# Autodesk Inventor assembly: Ventil
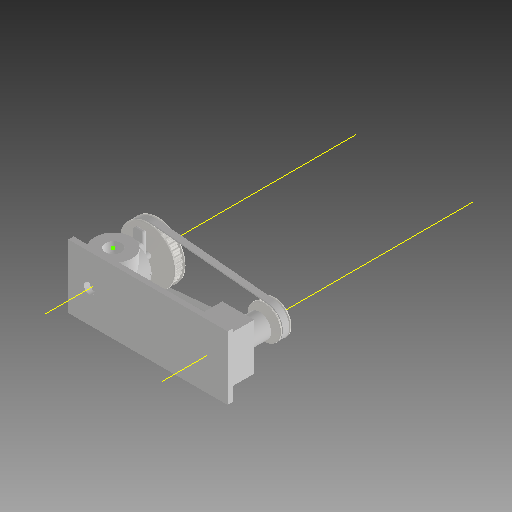
[picture p0: Inventor's stored thumbnail of the model, 512x512]
Saved by Autodesk Inventor 2021 (Build 250183000, 183)
## iProperties
Created: 2021-06-23
Part Number: Ventil
Document SubType Name: Assembly
Designer: stroh
Stock Number: Steuerbares Ventil
Author: stroh
## Documents named in this file (4)
- C:\Users\lukas\OneDrive - HTBLA Kaindorf\Diplomarbeit\Mechanik\InventorKonstruktion\Steuerbares Ventil\Ventil.iam
- C:\Users\lukas\OneDrive - HTBLA Kaindorf\Diplomarbeit\Mechanik\InventorKonstruktion\Steuerbares Ventil\Ventilrohr.ipt
- C:\Users\lukas\OneDrive - HTBLA Kaindorf\Diplomarbeit\Mechanik\InventorKonstruktion\Steuerbares Ventil\Ventilregler.ipt
- C:\Users\lukas\OneDrive - HTBLA Kaindorf\Diplomarbeit\Mechanik\InventorKonstruktion\Steuerbares Ventil\Ventil\Konstruktions-Assistent\Übertragung des Zahnriemens5.iam
## Components (3 placed, 3 different names)
1. Ventilrohr:1 — Einfügen:1
2. Ventilregler:1 — Einfügen:1
3. Übertragung des Zahnriemens:1 [sub-assembly]
## Relationships (1: Insert 1)
- Einfügen:1 [Insert]: Ventilrohr:1 ↔ Ventilregler:1
